# Autodesk Inventor assembly: model
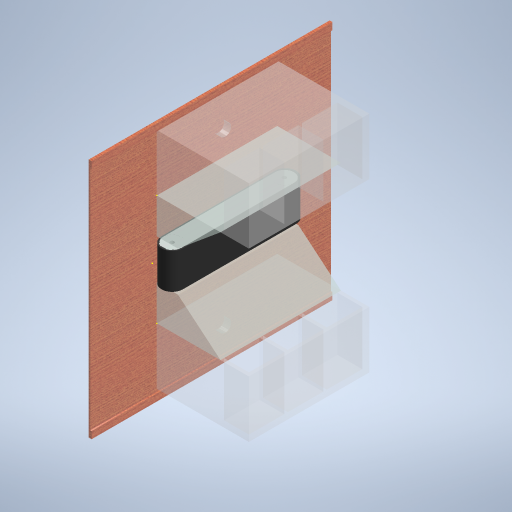
[picture p0: Inventor's stored thumbnail of the model, 512x512]
Saved by Autodesk Inventor 2023.1 (Build 271208000, 208)
## iProperties
Created: 2022-07-17
Part Number: model
Document SubType Name: Assembly
Designer: chand
Author: chand
## Documents named in this file (13)
- E:\exploration\model.iam
- E:\exploration\con.ipt
- E:\exploration\roller.ipt
- E:\exploration\Part1_MIR.ipt
- E:\exploration\slide_MIR.ipt
- E:\exploration\Part9.ipt
- E:\exploration\Part9_MIR.ipt
- E:\exploration\Part9_MIR1.ipt
- E:\exploration\Part19.ipt
- E:\exploration\Part1_MIR_MIR.ipt
- E:\exploration\slide_MIR_MIR.ipt
- E:\exploration\roller_MIR.ipt
- E:\exploration\Part9_MIR1_MIR.ipt
## Components (12 placed, 12 different names)
1. con:1 — Cylindrical:1, Mate:9, Mate:10, Mate:11, Rigid:1
2. Part1_MIR:1 — Mate:6, Mate:7, Mate:8, Mate:16, Mate:17, Mate:18, Mate:19, Mate:20
3. slide_MIR:1 — Mate:6, Mate:7, Mate:8, Mate:16
4. roller:1 — Cylindrical:1, Mate:11, Mate:12, Mate:15
5. Part9:1 — Mate:9, Mate:10, Mate:12
6. Part9_MIR1:1 — Mate:15
7. Part19:1 — Rigid:1, Mate:17, Mate:18, Mate:19, Mate:20
8. Part1_MIR_MIR:1 — Mate:21, Mate:22, Mate:23, Mate:24
9. slide_MIR_MIR:1 — Mate:21, Mate:22, Mate:23, Mate:24
10. roller_MIR:1 — Mate:25, Mate:26
11. Part9_MIR:1 — Mate:25
12. Part9_MIR1_MIR:1 — Mate:26
## Relationships (21: Mate 19, CylindricalJoint 1, WeldJoint 1)
- Mate:6: Part1_MIR:1 ↔ slide_MIR:1
- Mate:7: Part1_MIR:1 ↔ slide_MIR:1
- Mate:8: Part1_MIR:1 ↔ slide_MIR:1
- Cylindrical:1: con:1 ↔ roller:1
- Mate:9: con:1 ↔ Part9:1
- Mate:10: con:1 ↔ Part9:1
- Mate:11: con:1 ↔ roller:1
- Mate:12: roller:1 ↔ Part9:1
- Mate:15: roller:1 ↔ Part9_MIR1:1
- Mate:16: Part1_MIR:1 ↔ slide_MIR:1
- Rigid:1 [WeldJoint]: con:1 ↔ Part19:1
- Mate:17: Part1_MIR:1 ↔ Part19:1
- Mate:18: Part1_MIR:1 ↔ Part19:1
- Mate:19: Part1_MIR:1 ↔ Part19:1
- Mate:20 (238.633 mm): Part1_MIR:1 ↔ Part19:1
- Mate:21: Part1_MIR_MIR:1 ↔ slide_MIR_MIR:1
- Mate:22: Part1_MIR_MIR:1 ↔ slide_MIR_MIR:1
- Mate:23: Part1_MIR_MIR:1 ↔ slide_MIR_MIR:1
- Mate:24: Part1_MIR_MIR:1 ↔ slide_MIR_MIR:1
- Mate:25: roller_MIR:1 ↔ Part9_MIR:1
- Mate:26: roller_MIR:1 ↔ Part9_MIR1_MIR:1
